# Autodesk Inventor assembly: Satellite Gauche
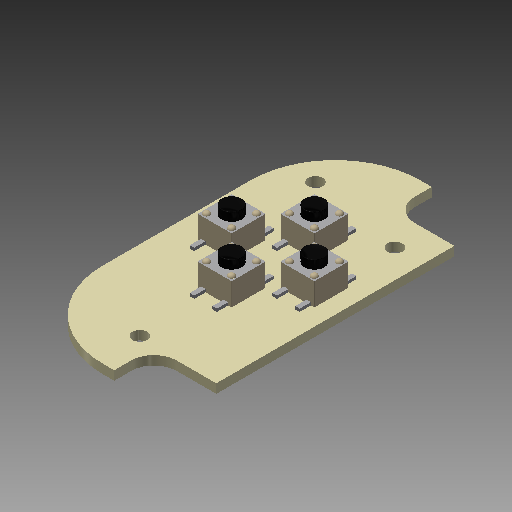
[picture p0: Inventor's stored thumbnail of the model, 512x512]
Saved by Autodesk Inventor 2019 (Build 230136000, 136)
## iProperties
Created: 2018-06-08
Part Number: Satellite Gauche
Material: Générique
Document SubType Name: Assembly
Designer: dimercur
Author: dimercur
## Documents named in this file (3)
- D:\Users\dimercur\Documents locaux\Travail\git\arm-ada-ng\hardware\Box\Satellite Gauche.iam
- D:\Users\dimercur\Documents locaux\Travail\git\arm-ada-ng\hardware\Box\PCB Gauche.ipt
- D:\Users\dimercur\Documents locaux\Travail\git\arm-ada-ng\hardware\Box\Touch Button.ipt
## Components (5 placed, 2 different names)
1. PCB Gauche:1 — Placage:1, Placage:2, Placage:3, Placage:4, Placage:5, Placage:6, Placage:7, Placage:8, Placage:9, Placage:10, Placage:11
2. Touch Button:1 — Placage:4, Placage:7, Placage:8, Placage:12
3. Touch Button:2 — Placage:2, Placage:9, Placage:12
4. Touch Button:3 — Placage:3, Placage:5, Placage:6
5. Touch Button:4 — Placage:1, Placage:10, Placage:11
## Relationships (12: Mate 12)
- Placage:1 [Mate]: PCB Gauche:1 ↔ Touch Button:4
- Placage:2 [Mate]: PCB Gauche:1 ↔ Touch Button:2
- Placage:3 [Mate]: PCB Gauche:1 ↔ Touch Button:3
- Placage:4 [Mate]: PCB Gauche:1 ↔ Touch Button:1
- Placage:5 [Mate] (10.25 mm): PCB Gauche:1 ↔ Touch Button:3
- Placage:6 [Mate] (8.45 mm): PCB Gauche:1 ↔ Touch Button:3
- Placage:7 [Mate] (17.55 mm): PCB Gauche:1 ↔ Touch Button:1
- Placage:8 [Mate] (15.75 mm): PCB Gauche:1 ↔ Touch Button:1
- Placage:9 [Mate] (15.75 mm): PCB Gauche:1 ↔ Touch Button:2
- Placage:10 [Mate] (10.25 mm): PCB Gauche:1 ↔ Touch Button:4
- Placage:11 [Mate] (23.05 mm): PCB Gauche:1 ↔ Touch Button:4
- Placage:12 [Mate] (8.6 mm): Touch Button:1 ↔ Touch Button:2
